# Autodesk Inventor assembly: EpoxyFitThroughKF16_Assembly
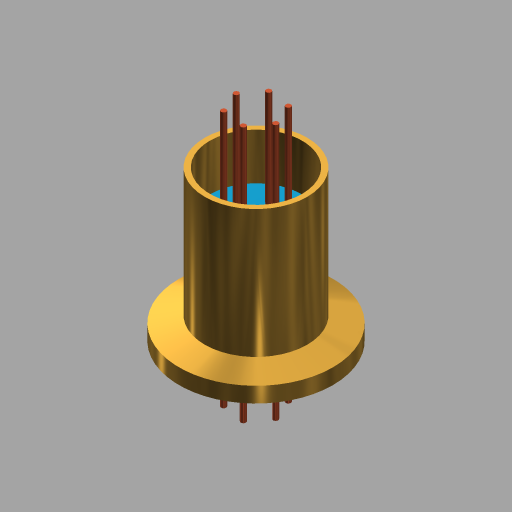
[picture p0: Inventor's stored thumbnail of the model, 512x512]
Saved by Autodesk Inventor 2024 (Build 280153020, 153B)
## iProperties
Created: 2023-10-02
Part Number: EpoxyFitThroughKF16_Assembly
Document SubType Name: Assembly
Designer: schanen
Author: schanen
## Documents named in this file (4)
- C:\Users\schanen\Documents\Inventor\he4inserts\EpoxyFitThroughKF16_Assembly.iam
- C:\Users\schanen\Documents\Inventor\he4inserts\EpoxyFitThroughKF16.ipt
- C:\Users\schanen\Documents\Inventor\he4inserts\EpoxyFitThroughKF16_mask.ipt
- C:\Users\schanen\Documents\Inventor\he4inserts\EpoxyFitThroughKF16_wire.ipt
## Components (8 placed, 3 different names)
1. EpoxyFitThroughKF16:1 — Mate:1, Mate:2, Flush:1
2. EpoxyFitThroughKF16_mask:1 — Mate:1, Mate:2, Mate:3
3. EpoxyFitThroughKF16_wire:1 — Mate:3, Flush:1
4. EpoxyFitThroughKF16_wire:2
5. EpoxyFitThroughKF16_wire:3
6. EpoxyFitThroughKF16_wire:4
7. EpoxyFitThroughKF16_wire:5
8. EpoxyFitThroughKF16_wire:6
## Component patterns: (6 elements, first: EpoxyFitThroughKF16_wire:1)
## Relationships (4: Mate 3, Flush 1)
- Mate:1: EpoxyFitThroughKF16:1 ↔ EpoxyFitThroughKF16_mask:1
- Mate:2: EpoxyFitThroughKF16:1 ↔ EpoxyFitThroughKF16_mask:1
- Mate:3: EpoxyFitThroughKF16_mask:1 ↔ EpoxyFitThroughKF16_wire:1
- Flush:1 (-10 mm): EpoxyFitThroughKF16:1 ↔ EpoxyFitThroughKF16_wire:1
